# Autodesk Inventor assembly: plate
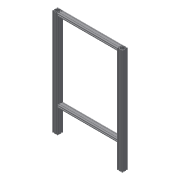
[picture p0: Inventor's stored thumbnail of the model, 180x180]
Saved by Autodesk Inventor 2018 (Build 220112000, 112)
## iProperties
Created: 2018-01-07
Part Number: plate
Document SubType Name: Assembly
Designer: sawaiz
Author: sawaiz
## Documents named in this file (3)
- C:\Users\sawaiz\OneDrive\personal\berlin\Move\larkspur\kitchen\frame\extrusions\plate.iam
- C:\Users\sawaiz\OneDrive\personal\berlin\Move\larkspur\kitchen\frame\extrusions\HFS5-4040-800.ipt
- C:\Users\sawaiz\OneDrive\personal\berlin\Move\larkspur\kitchen\frame\extrusions\HFS5-2040-450.ipt
## Components (4 placed, 2 different names)
1. HFS5-4040-800:1 — Flush:1, Flush:2, Mate:1, Mate:2, Flush:3, Flush:4, Flush:5, Symmetry:1, Symmetry:2, Symmetry:3
2. HFS5-4040-800:2 — Flush:1, Flush:2, Mate:3, Symmetry:1, Symmetry:2, Symmetry:3, Mate:4
3. HFS5-2040-450:1 — Mate:2, Flush:3, Flush:5, Mate:3
4. HFS5-2040-450:2 — Mate:1, Flush:4, Mate:4
## Relationships (12: Flush 5, Mate 4, Symmetry 3)
- Flush:1: HFS5-4040-800:1 ↔ HFS5-4040-800:2
- Flush:2: HFS5-4040-800:1 ↔ HFS5-4040-800:2
- Mate:1: HFS5-4040-800:1 ↔ HFS5-2040-450:2
- Mate:2: HFS5-4040-800:1 ↔ HFS5-2040-450:1
- Flush:3: HFS5-4040-800:1 ↔ HFS5-2040-450:1
- Flush:4: HFS5-4040-800:1 ↔ HFS5-2040-450:2
- Flush:5: HFS5-4040-800:1 ↔ HFS5-2040-450:1
- Mate:3: HFS5-4040-800:2 ↔ HFS5-2040-450:1
- Symmetry:1: HFS5-4040-800:1 ↔ HFS5-4040-800:2
- Symmetry:2: HFS5-4040-800:1 ↔ HFS5-4040-800:2
- Symmetry:3: HFS5-4040-800:1 ↔ HFS5-4040-800:2
- Mate:4 (-200 mm): HFS5-4040-800:2 ↔ HFS5-2040-450:2
